# Autodesk Inventor assembly: wafel_rev4
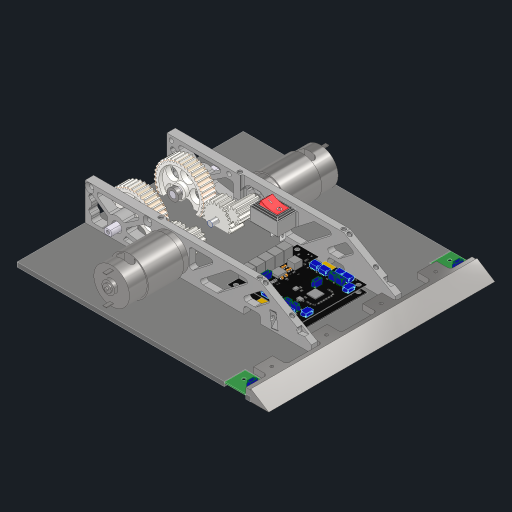
[picture p0: Inventor's stored thumbnail of the model, 512x512]
Saved by Autodesk Inventor 2023 (Build 270158000, 158)
## iProperties
Created: 2024-05-25
Part Number: wafel_rev4
Document SubType Name: Assembly
Designer: szymo
Mass: 910.827 g
Surface Area: 2620.28 cm^2
Volume: 529.707 cm^3
Density: 1.71949 g/cm^3
Author: szymo
## iProperties of the stored document TFMINI_S_UART.ipt
Created: 2023-12-04
Part Number: TFMINI S UART
Material: Generic
Description: STEP AP214
Document SubType Name: Modeling
Designer: mateu
Density: 1 g/cm^3
Appearance: Default
Mass: 6.04913 g
Surface Area: 27.6076 cm^2
Volume: 6.04913 cm^3
Sending System: SolidWorks 2016
Preprocessor: SwSTEP 2.0
Title: TFMINI S UART.STEP
Author: USER
Revision Number: ANY
## Documents named in this file (26)
- D:\roboilo\robots\codename wafel - australia\3d_parts\rev4\wafel_rev4.iam
- **D:\roboilo\robots\codename wafel - australia\3d_parts\rev4\wafel_rev4.iam*LocalDocs*xAaaaqfaaAaaaaaaaAaaaqmipQa*TFMINI_S_UART.ipt
- D:\roboilo\robots\codename wafel - australia\3d_parts\rev4\128x32-OLED.ipt
- D:\roboilo\robots\codename wafel - australia\3d_parts\rev4\interface_board.ipt
- D:\roboilo\robots\codename wafel - australia\3d_parts\rev4\KTIR-Board.ipt
- D:\roboilo\robots\codename wafel - australia\3d_parts\rev4\motor_w_gear.iam
- D:\roboilo\robots\codename wafel - australia\3d_parts\rev4\plog.ipt
- D:\roboilo\robots\codename wafel - australia\3d_parts\rev4\smolgear_shaft.ipt
- D:\roboilo\robots\codename wafel - australia\3d_parts\rev4\stack.iam
- D:\roboilo\robots\codename wafel - australia\3d_parts\rev4\Switch.ipt
- D:\roboilo\robots\codename wafel - australia\3d_parts\rev4\wheel_axle.iam
- D:\roboilo\robots\codename wafel - australia\3d_parts\rev4\Design Accelerator\smolGear.iam
- D:\roboilo\robots\codename wafel - australia\3d_parts\rev4\lipo3s650mah.ipt
- D:\roboilo\robots\codename wafel - australia\3d_parts\rev4\lipo2s450mah.ipt
- D:\roboilo\robots\codename wafel - australia\3d_parts\rev4\base.ipt
- D:\roboilo\robots\codename wafel - australia\3d_parts\rev4\side_r.ipt
- D:\roboilo\robots\codename wafel - australia\3d_parts\rev4\gaerHold_r.ipt
- D:\roboilo\robots\codename wafel - australia\3d_parts\rev4\side_r_MIR.ipt
- D:\roboilo\robots\codename wafel - australia\3d_parts\rev4\gaerHold_r_MIR.ipt
- D:\roboilo\robots\codename wafel - australia\3d_parts\rev4\blank_side_r.ipt
- D:\roboilo\robots\codename wafel - australia\3d_parts\rev4\blank_side_r_MIR.ipt
- D:\roboilo\robots\codename wafel - australia\3d_parts\rev4\wheeel_prep.ipt
- D:\roboilo\robots\codename wafel - australia\3d_parts\rev4\back.ipt
- D:\roboilo\robots\codename wafel - australia\3d_parts\rev4\ceil.ipt
- D:\roboilo\robots\codename wafel - australia\3d_parts\rev4\front.ipt
- D:\roboilo\robots\codename wafel - australia\3d_parts\rev4\TFMINI_S_UART.ipt
## Components (32 placed, 24 different names)
1. base:1 — Mate:3, Mate:4, Flush:5, Tangent:1, Tangent:2, Angle:2, Tangent:8, Tangent:10, Mate:5, Mate:6, Mate:9, Mate:10, Mate:12, Mate:13, Angle:6, Mate:14, Mate:15, Tangent:11, Tangent:12, Tangent:13, Tangent:14, Flush:18, Mate:19, Mate:20, Mate:21, Mate:22, Flush:19, Flush:20, Flush:21, Flush:23, Flush:24
2. plog:1 — Mate:3, Mate:4, Flush:5, Flush:10, Angle:1, Angle:3, Angle:4, Flush:11, Mate:11, Angle:5, Angle:7, Angle:8, Mate:16, Mate:17, Flush:22, Flush:39
3. side_r:1 — Flush:14, Flush:16, Mate:27, Flush:25, Flush:26, Flush:38, Mate:24
4. gaerHold_r:1 — Flush:18
5. blank_side_r:1 — Flush:22, Flush:23, Flush:24, Mate:29, Flush:40, Flush:28
6. gaerHold_r_MIR:1
7. side_r_MIR:1 — Mate:28, Flush:34, Mate:33, Mate:34, Flush:35, Mate:26
8. blank_side_r_MIR:1 — Mate:31, Flush:31, Flush:32, Flush:33, Flush:37
9. back:1 — Flush:27
10. stack:1 [sub-assembly] — Flush:10, Mate:5, Mate:7, Mate:8, Mate:11
11. motor_w_gear:1 [sub-assembly] — Tangent:1, Angle:2, Flush:8, Flush:9, Tangent:3, Mate:7, Tangent:11, Flush:14, Flush:16
12. wheel_axle:1 [sub-assembly] — Flush:9, Tangent:4, Tangent:10, Angle:3, Mate:10, Mate:23
13. smolGear:1 [sub-assembly] — Mate:1, Flush:8, Tangent:3, Tangent:4, Flush:13
14. smolgear_shaft:1 — Mate:1, Flush:13, Tangent:14
15. motor_w_gear:2 [sub-assembly] — Tangent:2, Angle:1, Flush:6, Flush:7, Tangent:5, Mate:8, Tangent:12
16. wheel_axle:2 [sub-assembly] — Flush:7, Tangent:6, Tangent:8, Angle:4, Mate:9, Mate:25
17. smolGear:2 [sub-assembly] — Mate:2, Flush:6, Tangent:5, Tangent:6, Flush:12
18. smolgear_shaft:2 — Mate:2, Flush:12, Tangent:13
19. lipo3s650mah:1 — Mate:15
20. lipo2s450mah:1 — Flush:11, Mate:6, Flush:21, Flush:27
21. lipo3s650mah:2 — Mate:14
22. TFMINI_S_UART:2 — Mate:12, Angle:5, Angle:7, Mate:17, Mate:28
23. TFMINI_S_UART:1 — Mate:13, Angle:6, Angle:8, Mate:16, Mate:27, Flush:25, Flush:26
24. KTIR-Board:1 — Mate:21, Mate:22, Flush:20
25. KTIR-Board:2 — Mate:19, Mate:20, Flush:19
26. 128x32-OLED:1 — Mate:31, Flush:31, Flush:32, Flush:33, Flush:37
27. interface_board:1 — Mate:29, Flush:40, Flush:28
28. Switch:1 — Flush:34, Mate:33, Mate:34, Flush:35
29. wheeel_prep:1 — Mate:23, Mate:24
30. wheeel_prep:2 — Mate:25, Mate:26
31. ceil:1 — Flush:38
32. front:1 — Flush:39
## Relationships (82: Mate 31, Flush 31, Tangent 12, Angle 8)
- Mate:1: smolGear:1 ↔ smolgear_shaft:1
- Mate:2: smolGear:2 ↔ smolgear_shaft:2
- Mate:3: base:1 ↔ plog:1
- Mate:4: base:1 ↔ plog:1
- Flush:5: base:1 ↔ plog:1
- Tangent:1: base:1 ↔ motor_w_gear:1
- Tangent:2: base:1 ↔ motor_w_gear:2
- Angle:1 (0 deg): plog:1 ↔ motor_w_gear:2
- Angle:2 (0 deg): base:1 ↔ motor_w_gear:1
- Flush:6: motor_w_gear:2 ↔ smolGear:2
- Flush:7: motor_w_gear:2 ↔ wheel_axle:2
- Flush:8: motor_w_gear:1 ↔ smolGear:1
- Flush:9: motor_w_gear:1 ↔ wheel_axle:1
- Tangent:3: motor_w_gear:1 ↔ smolGear:1
- Tangent:4: wheel_axle:1 ↔ smolGear:1
- Tangent:5: motor_w_gear:2 ↔ smolGear:2
- Tangent:6: wheel_axle:2 ↔ smolGear:2
- Tangent:8 (4 mm): base:1 ↔ wheel_axle:2
- Tangent:10 (4 mm): base:1 ↔ wheel_axle:1
- Flush:10 (61.5 mm): plog:1 ↔ stack:1
- Mate:5: base:1 ↔ stack:1
- Angle:3 (0 deg): plog:1 ↔ wheel_axle:1
- Angle:4 (0 deg): plog:1 ↔ wheel_axle:2
- Flush:11 (82 mm): plog:1 ↔ lipo2s450mah:1
- Mate:6: base:1 ↔ lipo2s450mah:1
- Flush:12 (5.3 mm): smolGear:2 ↔ smolgear_shaft:2
- Flush:13 (-5.3 mm): smolGear:1 ↔ smolgear_shaft:1
- Mate:7 (8 mm): stack:1 ↔ motor_w_gear:1
- Mate:8 (8 mm): stack:1 ↔ motor_w_gear:2
- Mate:9 (-25 mm): base:1 ↔ wheel_axle:2
- Mate:10 (-25 mm): base:1 ↔ wheel_axle:1
- Mate:11 (10 mm): plog:1 ↔ stack:1
- Mate:12: base:1 ↔ TFMINI_S_UART:2
- Angle:5 (-7 deg): plog:1 ↔ TFMINI_S_UART:2
- Mate:13: base:1 ↔ TFMINI_S_UART:1
- Angle:6 (-7 deg): base:1 ↔ TFMINI_S_UART:1
- Angle:7 (180 deg): plog:1 ↔ TFMINI_S_UART:2
- Angle:8 (180 deg): plog:1 ↔ TFMINI_S_UART:1
- Mate:14: base:1 ↔ lipo3s650mah:2
- Mate:15: base:1 ↔ lipo3s650mah:1
- Tangent:11 (52.5 mm): base:1 ↔ motor_w_gear:1
- Tangent:12 (52.5 mm): base:1 ↔ motor_w_gear:2
- Tangent:13 (2.55 mm): base:1 ↔ smolgear_shaft:2
- Tangent:14 (2.55 mm): base:1 ↔ smolgear_shaft:1
- Mate:16 (22 mm): plog:1 ↔ TFMINI_S_UART:1
- Mate:17 (22 mm): plog:1 ↔ TFMINI_S_UART:2
- Flush:14: side_r:1 ↔ motor_w_gear:1
- Flush:16: side_r:1 ↔ motor_w_gear:1
- Flush:18: base:1 ↔ gaerHold_r:1
- Mate:19 (0.5 mm): base:1 ↔ KTIR-Board:2
- Mate:20 (0.5 mm): base:1 ↔ KTIR-Board:2
- Mate:21 (0.5 mm): base:1 ↔ KTIR-Board:1
- Mate:22 (0.5 mm): base:1 ↔ KTIR-Board:1
- Flush:19: base:1 ↔ KTIR-Board:2
- Flush:20: base:1 ↔ KTIR-Board:1
- Flush:21: base:1 ↔ lipo2s450mah:1
- Flush:22: plog:1 ↔ blank_side_r:1
- Flush:23: base:1 ↔ blank_side_r:1
- Flush:24: base:1 ↔ blank_side_r:1
- Mate:23: wheel_axle:1 ↔ wheeel_prep:1
- Mate:24 (1.5 mm): side_r:1 ↔ wheeel_prep:1
- Mate:25: wheel_axle:2 ↔ wheeel_prep:2
- Mate:26 (1.5 mm): side_r_MIR:1 ↔ wheeel_prep:2
- Mate:27: side_r:1 ↔ TFMINI_S_UART:1
- Mate:28: side_r_MIR:1 ↔ TFMINI_S_UART:2
- Flush:25: side_r:1 ↔ TFMINI_S_UART:1
- Flush:26 (28 mm): side_r:1 ↔ TFMINI_S_UART:1
- Flush:27: back:1 ↔ lipo2s450mah:1
- Mate:29: blank_side_r:1 ↔ interface_board:1
- Flush:40: blank_side_r:1 ↔ interface_board:1
- Flush:28: blank_side_r:1 ↔ interface_board:1
- Mate:31: blank_side_r_MIR:1 ↔ 128x32-OLED:1
- Flush:31 (3 mm): blank_side_r_MIR:1 ↔ 128x32-OLED:1
- Flush:32: blank_side_r_MIR:1 ↔ 128x32-OLED:1
- Flush:33 (-5.5 mm): blank_side_r_MIR:1 ↔ 128x32-OLED:1
- Flush:34 (2 mm): side_r_MIR:1 ↔ Switch:1
- Mate:33: side_r_MIR:1 ↔ Switch:1
- Mate:34 (-6 mm): side_r_MIR:1 ↔ Switch:1
- Flush:35: side_r_MIR:1 ↔ Switch:1
- Flush:37: blank_side_r_MIR:1 ↔ 128x32-OLED:1
- Flush:38: side_r:1 ↔ ceil:1
- Flush:39: plog:1 ↔ front:1
